# Autodesk Inventor assembly: Ribbon cable test
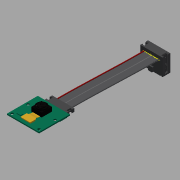
[picture p0: Inventor's stored thumbnail of the model, 180x180]
Saved by Autodesk Inventor 2017 (Build 210142000, 142)
## iProperties
Created: 2017-01-19
Part Number: Ribbon cable test
Document SubType Name: Assembly
Designer: qupec
Author: qupec
## Documents named in this file (5)
- C:\Users\qupec\Desktop\UMD Near Space\RockSat\Ribbon cable test.iam
- C:\Users\qupec\Desktop\UMD Near Space\RockSat\Pi Cam\RasPi_Camera.iam
- C:\Users\qupec\Desktop\UMD Near Space\RockSat\Ribbon Cable Connector-01.ipt
- C:\Users\qupec\Documents\Inventor\Content Center Files\R2017\en-US\Ribbon Cable Connector\Ribbon Cable Connector-01.ipt
- C:\Users\qupec\Desktop\UMD Near Space\RockSat\Ribbon cable test\AIP\Cable and Harness\Ribbon cable test.Harness3.iam
## Components (4 placed, 4 different names)
1. RasPi_Camera:1 [sub-assembly] — Mate:2, Flush:2
2. Ribbon Cable Connector-01:1 — Mate:2, Flush:1
3. Ribbon Cable Connector Ribbon Cable Connector-01:2 — Flush:1, Flush:2
4. Harness3 [sub-assembly]
## Relationships (3: Flush 2, Mate 1)
- Mate:2: RasPi_Camera:1 ↔ Ribbon Cable Connector-01:1
- Flush:1: Ribbon Cable Connector-01:1 ↔ Ribbon Cable Connector Ribbon Cable Connector-01:2
- Flush:2: RasPi_Camera:1 ↔ Ribbon Cable Connector Ribbon Cable Connector-01:2
